# Autodesk Inventor assembly: User Library-plastic bearings_igus nk02-40-2-610
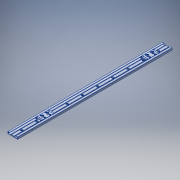
[picture p0: Inventor's stored thumbnail of the model, 180x180]
Saved by Autodesk Inventor 2018 (Build 220112000, 112)
## iProperties
Created: 2019-01-10
Part Number: User Library-plastic bearings_igus nk02-40-2-610
Description: STEP AP214
Document SubType Name: Assembly
Designer: maste
Sending System: SolidWorks 2018
Preprocessor: SwSTEP 2.0
Title: User Library-plastic bearings_igus nk02-40-2-610.STEP
Revision Number: ANY
## Documents named in this file (3)
- C:\Users\maste\OneDrive\Documents\GitHub\2019CAD\Drivebase but Calvin is a mad man\User Library-plastic bearings_igus nk02-40-2-610.iam
- C:\Users\maste\OneDrive\Documents\GitHub\2019CAD\Drivebase but Calvin is a mad man\User Library-plastic bearings_igus nk02-40-2-610_nk04-40_rail.ipt
- C:\Users\maste\OneDrive\Documents\GitHub\2019CAD\Drivebase but Calvin is a mad man\User Library-plastic bearings_igus nk02-40-2-610_nk04-40_carriage.ipt
## Components (3 placed, 3 different names)
1. User Library-plastic bearings_igus nk02-40-2-610_nk04-40_rail_1 — Mate:1, Mate:2, Mate:3, Mate:4
2. User Library-plastic bearings_igus nk02-40-2-610_nk04-40_carriage_2 — Mate:1, Mate:2
3. User Library-plastic bearings_igus nk02-40-2-610_nk04-40_carriage_3 — Mate:3, Mate:4
## Relationships (4: Mate 4)
- Mate:1: User Library-plastic bearings_igus nk02-40-2-610_nk04-40_rail_1 ↔ User Library-plastic bearings_igus nk02-40-2-610_nk04-40_carriage_2
- Mate:2: User Library-plastic bearings_igus nk02-40-2-610_nk04-40_rail_1 ↔ User Library-plastic bearings_igus nk02-40-2-610_nk04-40_carriage_2
- Mate:3: User Library-plastic bearings_igus nk02-40-2-610_nk04-40_rail_1 ↔ User Library-plastic bearings_igus nk02-40-2-610_nk04-40_carriage_3
- Mate:4: User Library-plastic bearings_igus nk02-40-2-610_nk04-40_rail_1 ↔ User Library-plastic bearings_igus nk02-40-2-610_nk04-40_carriage_3
